# Autodesk Inventor assembly: FinalRobot-ver1-1111-2021
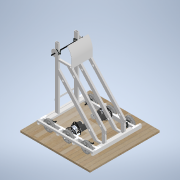
[picture p0: Inventor's stored thumbnail of the model, 180x180]
Saved by Autodesk Inventor 2020 (Build 240168000, 168)
## iProperties
Created: 2021-01-26
Part Number: FinalRobot-ver1-1111-2021
Document SubType Name: Assembly
Designer: Caitlin
Author: Caitlin
## Documents named in this file (5)
- D:\PHRC CADD 2021\PHRC CADD\2020 Infinite Recharge\2021 Infinite Recharge\FinalRobot-ver1-1111-2021.iam
- D:\PHRC CADD 2021\PHRC CADD\2020 Infinite Recharge\2021 Infinite Recharge\Chassis\Chassis-ver1-1111-2021.iam
- D:\PHRC CADD 2021\PHRC CADD\2020 Infinite Recharge\Platform.ver1-1111-2020.ipt
- D:\PHRC CADD 2021\PHRC CADD\2020 Infinite Recharge\Storage\Assemblies\StorageAssembly.ver4-1111-2020.iam
- D:\PHRC CADD 2021\PHRC CADD\2020 Infinite Recharge\Shooting\Assemblies\ShooterPrototype-ver2-1111-2019.iam
## Components (4 placed, 4 different names)
1. Chassis-ver1-1111-2021:1 [sub-assembly] — Mate:1, Angle:1, Flush:1, Flush:2, Mate:2, Mate:3, Mate:4, Mate:5, Mate:6, Flush:3
2. Platform.ver1-1111-2020:1 — Mate:1, Angle:1, Flush:1, Flush:2
3. StorageAssembly.ver4-1111-2020:1 [sub-assembly] — Mate:2, Mate:3, Mate:4
4. ShooterPrototype-ver2-1111-2019:1 [sub-assembly] — Mate:5, Mate:6, Flush:3
## Relationships (10: Mate 6, Flush 3, Angle 1)
- Mate:1 (47.625 mm): Chassis-ver1-1111-2021:1 ↔ Platform.ver1-1111-2020:1
- Angle:1 (0 deg): Chassis-ver1-1111-2021:1 ↔ Platform.ver1-1111-2020:1
- Flush:1 (152.4 mm): Chassis-ver1-1111-2021:1 ↔ Platform.ver1-1111-2020:1
- Flush:2 (114.3 mm): Chassis-ver1-1111-2021:1 ↔ Platform.ver1-1111-2020:1
- Mate:2: Chassis-ver1-1111-2021:1 ↔ StorageAssembly.ver4-1111-2020:1
- Mate:3: Chassis-ver1-1111-2021:1 ↔ StorageAssembly.ver4-1111-2020:1
- Mate:4: Chassis-ver1-1111-2021:1 ↔ StorageAssembly.ver4-1111-2020:1
- Mate:5: Chassis-ver1-1111-2021:1 ↔ ShooterPrototype-ver2-1111-2019:1
- Mate:6: Chassis-ver1-1111-2021:1 ↔ ShooterPrototype-ver2-1111-2019:1
- Flush:3: Chassis-ver1-1111-2021:1 ↔ ShooterPrototype-ver2-1111-2019:1
